# Autodesk Inventor assembly: Plataforma_equipada
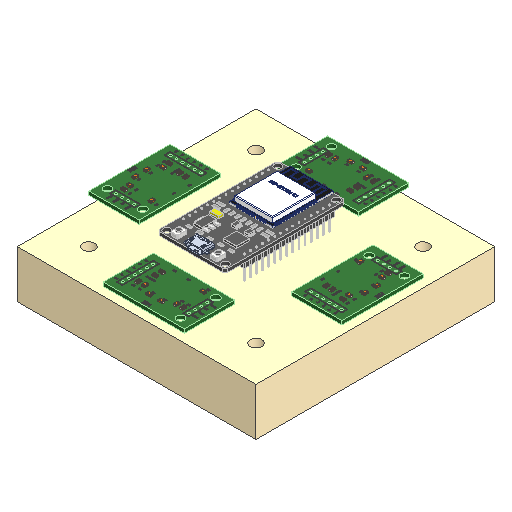
[picture p0: Inventor's stored thumbnail of the model, 512x512]
Saved by Autodesk Inventor 2026.1 (Build 301233000, 233)
## iProperties
Created: 2025-10-01
Part Number: Plataforma_equipada
Document SubType Name: Assembly
Designer: gianm
Author: gianm
## Documents named in this file (4)
- D:\Tesis\Modelo 3D\CAD\Plataforma_equipada.iam
- D:\Tesis\Modelo 3D\CAD\Plataforma.ipt
- D:\Tesis\Modelo 3D\CAD\Electronicos\hx711-breakout-board-1.snapshot.2\HX711 Breakout v8 ohne Pinheader\HX711 Breakout v8 ohne Pinheader\HX711 Breakout v8 ohne Pinheader.iam
- D:\Tesis\Modelo 3D\CAD\Electronicos\esp-32-1.snapshot.6\ESP-32_v1\ESP-32_v1\ESP-32_v1.iam
## Components (6 placed, 3 different names)
1. Plataforma:1 — Coincidencia:1, Coincidencia:2, Ángulo:1, Ángulo:2, Ángulo:3, Nivelación:1, Nivelación:2
2. ESP-32_v1:1 [sub-assembly]
3. HX711 Breakout v8 ohne Pinheader:1 [sub-assembly] — Nivelación:1, Nivelación:2
4. HX711 Breakout v8 ohne Pinheader:2 [sub-assembly]
5. HX711 Breakout v8 ohne Pinheader:3 [sub-assembly]
6. HX711 Breakout v8 ohne Pinheader:4 [sub-assembly]
## Component patterns: (4 elements, first: HX711 Breakout v8 ohne Pinheader:1)
## Relationships (12: Mate 7, Angle 3, Flush 2)
- Coincidencia:1 [Mate]: Plataforma:1
- Coincidencia:2 [Mate]: Plataforma:1
- Coincidencia:3 [Mate]
- Ángulo:1 [Angle] (0 deg): Plataforma:1
- Coincidencia:4 [Mate]
- Ángulo:2 [Angle] (0 deg): Plataforma:1
- Coincidencia:5 [Mate]
- Coincidencia:6 [Mate]
- Coincidencia:7 [Mate]
- Ángulo:3 [Angle] (0 deg): Plataforma:1
- Nivelación:1 [Flush]: Plataforma:1 ↔ HX711 Breakout v8 ohne Pinheader:1
- Nivelación:2 [Flush] (30 mm): Plataforma:1 ↔ HX711 Breakout v8 ohne Pinheader:1
